# Autodesk Inventor assembly: Baugruppe_Christian_Test
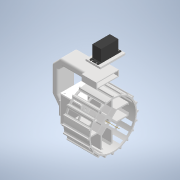
[picture p0: Inventor's stored thumbnail of the model, 180x180]
Saved by Autodesk Inventor 2021 (Build 250183000, 183)
## iProperties
Created: 2021-01-04
Part Number: Baugruppe_Christian_Test
Document SubType Name: Assembly
Designer: Ctroi
Mass: 279.93 g
Surface Area: 1178.31 cm^2
Volume: 279.93 cm^3
Density: 1 g/cm^3
Author: Ctroi
## Documents named in this file (8)
- G:\Roverprojekt\Github Projekt\Rover\Baugruppe_Christian_Test.iam
- G:\Roverprojekt\Github Projekt\Rover\Motorhalterung_v2.ipt
- G:\Roverprojekt\Github Projekt\Rover\Steppermotor.ipt
- G:\Roverprojekt\Github Projekt\Rover\Reifen_v2.ipt
- G:\Roverprojekt\Github Projekt\Rover\Verbindung_Motor_Servo_v2.ipt
- G:\Roverprojekt\Github Projekt\Rover\Motorhalterung_Klemme.ipt
- G:\Roverprojekt\Github Projekt\Rover\Servohalterung_v2.ipt
- G:\Roverprojekt\Github Projekt\Rover\Servo.ipt
## Components (7 placed, 7 different names)
1. Steppermotor:1 — Passend:1, Passend:2, Passend:3, Drehbar:1
2. Motorhalterung_v2:1 — Passend:1, Passend:2, Passend:3, Fluchtend:2, Passend:4, Passend:5
3. Motorhalterung_Klemme:1 — Fluchtend:2, Passend:4, Passend:5, Passend:6, Fluchtend:3, Passend:7
4. Reifen_v2:1 — Drehbar:1
5. Verbindung_Motor_Servo_v2:1 — Passend:6, Fluchtend:3, Passend:7
6. Servohalterung_v2:1 — Passend:8, Passend:9
7. Servo:1 — Passend:8, Passend:9
## Relationships (12: Mate 9, Flush 2, RevoluteJoint 1)
- Passend:1 [Mate]: Steppermotor:1 ↔ Motorhalterung_v2:1
- Passend:2 [Mate]: Steppermotor:1 ↔ Motorhalterung_v2:1
- Passend:3 [Mate]: Steppermotor:1 ↔ Motorhalterung_v2:1
- Fluchtend:2 [Flush]: Motorhalterung_v2:1 ↔ Motorhalterung_Klemme:1
- Passend:4 [Mate]: Motorhalterung_v2:1 ↔ Motorhalterung_Klemme:1
- Passend:5 [Mate]: Motorhalterung_v2:1 ↔ Motorhalterung_Klemme:1
- Drehbar:1 [RevoluteJoint] (-20 mm): Steppermotor:1 ↔ Reifen_v2:1
- Passend:6 [Mate]: Motorhalterung_Klemme:1 ↔ Verbindung_Motor_Servo_v2:1
- Fluchtend:3 [Flush]: Motorhalterung_Klemme:1 ↔ Verbindung_Motor_Servo_v2:1
- Passend:7 [Mate]: Motorhalterung_Klemme:1 ↔ Verbindung_Motor_Servo_v2:1
- Passend:8 [Mate]: Servohalterung_v2:1 ↔ Servo:1
- Passend:9 [Mate]: Servohalterung_v2:1 ↔ Servo:1
